# Autodesk Inventor assembly: extruder
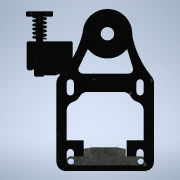
[picture p0: Inventor's stored thumbnail of the model, 180x180]
Saved by Autodesk Inventor 2020 (Build 240168000, 168)
## iProperties
Created: 2021-03-17
Part Number: extruder
Document SubType Name: Assembly
Designer: AOB
Mass: 29.4496 g
Surface Area: 141.694 cm^2
Volume: 20.1602 cm^3
Density: 1.46078 g/cm^3
Author: AOB
## Documents named in this file (3)
- C:\Users\marti\Documents\Inventor\ProjectBoron\ultimate boron\extruder.iam
- C:\Users\marti\Documents\Inventor\ProjectBoron\ultimate boron\motor mount2.ipt
- C:\Users\marti\Documents\Inventor\ProjectBoron\ultimate boron\tensioner.ipt
## Components (2 placed, 2 different names)
1. motor mount2:1 — Mate:1
2. tensioner:1 — Mate:1
## Relationships (1: Mate 1)
- Mate:1: motor mount2:1 ↔ tensioner:1
